# Autodesk Inventor assembly: outer case storage.p
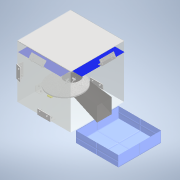
[picture p0: Inventor's stored thumbnail of the model, 180x180]
Saved by Autodesk Inventor 2021 (Build 250183000, 183)
## iProperties
Created: 2021-03-07
Part Number: outer case storage.p
Document SubType Name: Assembly
Designer: Spoorthi Honnalli
Author: Spoorthi Honnalli
## Documents named in this file (10)
- C:\Users\Spoorthi Honnalli\Downloads\outer case storage.p.iam
- C:\Users\Spoorthi Honnalli\3D Objects\outer case.p.ipt.iam
- C:\Users\Spoorthi Honnalli\3D Objects\storage.p1.iam
- C:\Users\Spoorthi Honnalli\3D Objects\dsk.ipt
- C:\Users\Spoorthi Honnalli\OneDrive\dc motor p.ipt
- C:\Users\Spoorthi Honnalli\3D Objects\pipe.ipt
- C:\Users\Spoorthi Honnalli\3D Objects\try.p.ipt
- C:\Users\Spoorthi Honnalli\3D Objects\lid.ipt
- C:\Users\Spoorthi Honnalli\3D Objects\sup.1p.ipt
- outer case.p.ipt
## Components (8 placed, 8 different names)
1. outer case.p.ipt:1 [sub-assembly]
2. storage.p1:1 [sub-assembly]
3. dsk:1 — Mate:1
4. dc motor p:1 — Mate:1, Mate:2
5. pipe:1
6. try.p:1
7. lid:1
8. sup.1p:1 — Mate:2
## Relationships (2: Mate 2)
- Mate:1: dsk:1 ↔ dc motor p:1
- Mate:2: dc motor p:1 ↔ sup.1p:1
